# Autodesk Inventor assembly: ASY PRS 940-20 charging hatch
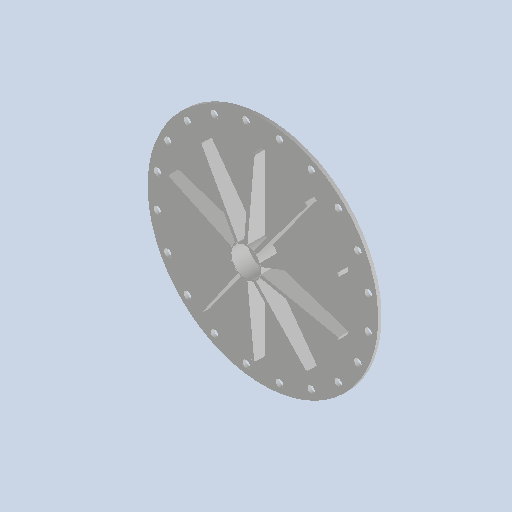
[picture p0: Inventor's stored thumbnail of the model, 512x512]
Saved by Autodesk Inventor 2025 (Build 290162010, 162A)
## iProperties
Created: 2025-04-22
Part Number: ASY PRS 940-20 charging hatch
Document SubType Name: Assembly
Designer: user
Mass: 9483.1 g
Surface Area: 9977.57 cm^2
Volume: 3616.18 cm^3
Density: 2.6224 g/cm^3
Author: user
## Documents named in this file (4)
- C:\Users\pokla\Documents\Inventor\PRS-Purovskii\Model\PRS-filter 940\ASY PRS 940-20 charging hatch.iam
- C:\Users\pokla\Documents\Inventor\PRS-Purovskii\Model\PRS-filter 940\PRS 940-21 charging hatch.ipt
- C:\Users\pokla\Documents\Inventor\PRS-Purovskii\Model\PRS-filter 940\PRS 940-23 charging hatch reinf 500mm.ipt
- C:\Users\pokla\Documents\Inventor\PRS-Purovskii\Model\PRS-filter 940\PRS 940-22 hatch tube 512mm.ipt
## Components (12 placed, 3 different names)
1. PRS 940-21 charging hatch.ipt:1 — Rigid:1, Flush:1
2. PRS 940-22 hatch tube 512mm.ipt:1 — Rigid:1
3. PRS 940-23 charging hatch reinf 500mm.ipt:1 — Mate:1, Flush:1, Mate:2, Mate:3
4. PRS 940-23 charging hatch reinf 500mm.ipt:2
5. PRS 940-23 charging hatch reinf 500mm.ipt:3
6. PRS 940-23 charging hatch reinf 500mm.ipt:4
7. PRS 940-23 charging hatch reinf 500mm.ipt:5
8. PRS 940-23 charging hatch reinf 500mm.ipt:6
9. PRS 940-23 charging hatch reinf 500mm.ipt:7
10. PRS 940-23 charging hatch reinf 500mm.ipt:8
11. PRS 940-23 charging hatch reinf 500mm.ipt:9
12. PRS 940-23 charging hatch reinf 500mm.ipt:10
## Component patterns: (10 elements, first: PRS 940-23 charging hatch reinf 500mm.ipt:1)
## Relationships (5: Mate 3, WeldJoint 1, Flush 1)
- Rigid:1 [WeldJoint]: PRS 940-21 charging hatch.ipt:1 ↔ PRS 940-22 hatch tube 512mm.ipt:1
- Mate:1: PRS 940-23 charging hatch reinf 500mm.ipt:1
- Flush:1: PRS 940-21 charging hatch.ipt:1 ↔ PRS 940-23 charging hatch reinf 500mm.ipt:1
- Mate:2: PRS 940-23 charging hatch reinf 500mm.ipt:1
- Mate:3: PRS 940-23 charging hatch reinf 500mm.ipt:1
